# Autodesk Inventor assembly: support_arriere
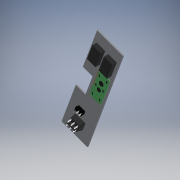
[picture p0: Inventor's stored thumbnail of the model, 180x180]
Saved by Autodesk Inventor 2017 (Build 210142000, 142)
## iProperties
Created: 2017-04-21
Part Number: support_arriere
Document SubType Name: Assembly
Designer: franc
Author: franc
## Documents named in this file (6)
- C:\Users\franc\Desktop\EsialRobotik\Mecanique\robot-2017\support_arriere.iam
- C:\Users\franc\Desktop\EsialRobotik\Mecanique\robot-2017\base_support_arriere.ipt
- C:\Users\franc\Desktop\EsialRobotik\Mecanique\utils\Voltmetre\VDC1.ipt
- C:\Users\franc\Desktop\EsialRobotik\Mecanique\utils\LCD\lcd_1602.iam
- C:\Users\franc\Desktop\EsialRobotik\Mecanique\utils\Interrupteur\Switch double\switch-double.ipt
- C:\Users\franc\Desktop\EsialRobotik\Mecanique\utils\Interrupteur\Switch simple\EnsamblajeSwitch.iam
## Components (6 placed, 5 different names)
1. base_support_arriere:1 — Mate:1, Mate:2, Mate:3, Mate:4, Mate:5, Mate:6, Mate:7, Mate:8, Mate:9, Mate:10, Mate:11, Mate:12, Mate:13, Mate:15, Mate:16
2. VDC1:1 — Mate:1, Mate:2, Mate:3
3. VDC1:2 — Mate:4, Mate:5, Mate:6
4. lcd_1602:1 [sub-assembly] — Mate:7, Mate:8, Mate:9
5. switch-double:1 — Mate:13, Mate:15, Mate:16
6. EnsamblajeSwitch:1 [sub-assembly] — Mate:10, Mate:11, Mate:12
## Relationships (15: Mate 15)
- Mate:1: base_support_arriere:1 ↔ VDC1:1
- Mate:2: base_support_arriere:1 ↔ VDC1:1
- Mate:3: base_support_arriere:1 ↔ VDC1:1
- Mate:4: base_support_arriere:1 ↔ VDC1:2
- Mate:5: base_support_arriere:1 ↔ VDC1:2
- Mate:6: base_support_arriere:1 ↔ VDC1:2
- Mate:7: base_support_arriere:1 ↔ lcd_1602:1
- Mate:8: base_support_arriere:1 ↔ lcd_1602:1
- Mate:9: base_support_arriere:1 ↔ lcd_1602:1
- Mate:10: base_support_arriere:1 ↔ EnsamblajeSwitch:1
- Mate:11: base_support_arriere:1 ↔ EnsamblajeSwitch:1
- Mate:12: base_support_arriere:1 ↔ EnsamblajeSwitch:1
- Mate:13: base_support_arriere:1 ↔ switch-double:1
- Mate:15: base_support_arriere:1 ↔ switch-double:1
- Mate:16 (2 mm): base_support_arriere:1 ↔ switch-double:1
